# Autodesk Inventor assembly: suspension_one_side
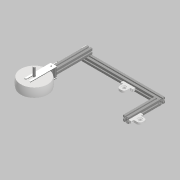
[picture p0: Inventor's stored thumbnail of the model, 180x180]
Saved by Autodesk Inventor 2021.2 (Build 252289000, 289)
## iProperties
Created: 2021-05-27
Part Number: suspension_one_side
Document SubType Name: Assembly
Designer: gisen
Author: gisen
## Documents named in this file (7)
- C:\Users\gisen\workspace\beetle_inventor_model\suspension\rocker_left.iam
- C:\Users\gisen\workspace\beetle_inventor_model\suspension\C-BGHKA6902ZZ-30\C-BGHKA6902ZZ-30.iam
- C:\Users\gisen\workspace\beetle_inventor_model\suspension\AFS-3030-435.ipt
- C:\Users\gisen\workspace\beetle_inventor_model\suspension\AFS-3030-200.ipt
- C:\Users\gisen\workspace\beetle_inventor_model\suspension\wheel_with_mounts.iam
- C:\Users\gisen\workspace\beetle_inventor_model\suspension\AFS-3030-174.ipt
- C:\Users\gisen\workspace\beetle_inventor_model\suspension\rocker_frame_mount.ipt
## Components (7 placed, 6 different names)
1. C-BGHKA6902ZZ-30:1 [sub-assembly] — メイト:5, メイト:18
2. AFS-3030-435:1 — メイト:5, フラッシュ:6, フラッシュ:7, メイト:6, メイト:8, メイト:9, メイト:10, メイト:11, メイト:15, フラッシュ:9, メイト:17
3. AFS-3030-174:1 — フラッシュ:6, フラッシュ:7, メイト:6, メイト:18, メイト:19
4. rocker_frame_mount:1 — メイト:8, メイト:16, メイト:17
5. C-BGHKA6902ZZ-30:2 [sub-assembly] — メイト:9, メイト:10, メイト:11, メイト:19
6. AFS-3030-200:1 — メイト:13, フラッシュ:8, メイト:14, メイト:15, フラッシュ:9, メイト:16
7. wheel_with_mounts:1 [sub-assembly] — メイト:13, フラッシュ:8, メイト:14, フラッシュ:10
## Relationships (18: Mate 13, Flush 5)
- メイト:5 [Mate] (-15 mm): C-BGHKA6902ZZ-30:1 ↔ AFS-3030-435:1
- フラッシュ:6 [Flush]: AFS-3030-435:1 ↔ AFS-3030-174:1
- フラッシュ:7 [Flush]: AFS-3030-435:1 ↔ AFS-3030-174:1
- メイト:6 [Mate]: AFS-3030-435:1 ↔ AFS-3030-174:1
- メイト:8 [Mate]: AFS-3030-435:1 ↔ rocker_frame_mount:1
- メイト:9 [Mate] (-15 mm): AFS-3030-435:1 ↔ C-BGHKA6902ZZ-30:2
- メイト:10 [Mate] (-15 mm): AFS-3030-435:1 ↔ C-BGHKA6902ZZ-30:2
- メイト:11 [Mate]: AFS-3030-435:1 ↔ C-BGHKA6902ZZ-30:2
- メイト:13 [Mate]: AFS-3030-200:1 ↔ wheel_with_mounts:1
- フラッシュ:8 [Flush]: AFS-3030-200:1 ↔ wheel_with_mounts:1
- メイト:14 [Mate]: AFS-3030-200:1 ↔ wheel_with_mounts:1
- メイト:15 [Mate] (3 mm): AFS-3030-435:1 ↔ AFS-3030-200:1
- フラッシュ:9 [Flush]: AFS-3030-435:1 ↔ AFS-3030-200:1
- メイト:16 [Mate]: rocker_frame_mount:1 ↔ AFS-3030-200:1
- メイト:17 [Mate]: AFS-3030-435:1 ↔ rocker_frame_mount:1
- メイト:18 [Mate]: C-BGHKA6902ZZ-30:1 ↔ AFS-3030-174:1
- フラッシュ:10 [Flush]: wheel_with_mounts:1
- メイト:19 [Mate] (150 mm): AFS-3030-174:1 ↔ C-BGHKA6902ZZ-30:2
